# Autodesk Inventor assembly: chassis_assembly_modified
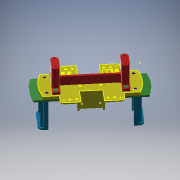
[picture p0: Inventor's stored thumbnail of the model, 180x180]
Saved by Autodesk Inventor 2017 SP1 (Build 210196100, 196)
## iProperties
Part Number: chassis_assembly_modified
Material: Générique
Document SubType Name: Assembly
Designer: tmonglon
Author: tmonglon
## Documents named in this file (5)
- D:\Inventor\Ahmet\mai_2017\chassis_assembly_modified.iam
- D:\Inventor\Ahmet\mai_2017\red_part_modified.ipt
- D:\Inventor\Ahmet\mai_2017\yellow_part_modified.ipt
- D:\Inventor\Ahmet\mai_2017\green_part_modified.ipt
- D:\Inventor\Ahmet\mai_2017\blue_part_modified.ipt
## Components (6 placed, 4 different names)
1. red_part_modified:1 — Logement:1, Placage:1
2. yellow_part_modified:1 — Logement:1, Placage:1, Logement:2, Logement:3, Logement:4, Logement:5, Logement:6, Logement:8, Logement:9
3. green_part_modified:1 — Logement:2, Logement:5, Logement:7
4. green_part_modified:2 — Logement:3, Logement:4
5. blue_part_modified:1 — Logement:6, Logement:7
6. blue_part_modified:2 — Logement:8, Logement:9
## Relationships (10: Insert 9, Mate 1)
- Logement:1 [Insert]: red_part_modified:1 ↔ yellow_part_modified:1
- Placage:1 [Mate]: red_part_modified:1 ↔ yellow_part_modified:1
- Logement:2 [Insert]: yellow_part_modified:1 ↔ green_part_modified:1
- Logement:3 [Insert]: yellow_part_modified:1 ↔ green_part_modified:2
- Logement:4 [Insert]: yellow_part_modified:1 ↔ green_part_modified:2
- Logement:5 [Insert]: yellow_part_modified:1 ↔ green_part_modified:1
- Logement:6 [Insert]: yellow_part_modified:1 ↔ blue_part_modified:1
- Logement:7 [Insert]: green_part_modified:1 ↔ blue_part_modified:1
- Logement:8 [Insert]: yellow_part_modified:1 ↔ blue_part_modified:2
- Logement:9 [Insert]: yellow_part_modified:1 ↔ blue_part_modified:2
